# Autodesk Inventor assembly: Topic 15-3_凸輪動力學模擬_test_5
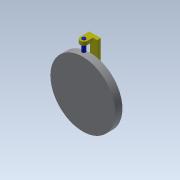
[picture p0: Inventor's stored thumbnail of the model, 180x180]
Saved by Autodesk Inventor 2022 (Build 260153000, 153)
## iProperties
Created: 2020-03-26
Part Number: Topic 15-3_凸輪動力學模擬_test_5
Document SubType Name: Assembly
Designer: Kuan-Lun Hsu
Author: Kuan-Lun Hsu
## Documents named in this file (5)
- C:\Users\Johnny Jou\Documents\GitHub\Special-project\CamSimulaiton\Topic 15-3_凸輪動力學模擬_test_5.iam
- C:\Users\Johnny Jou\Documents\GitHub\Special-project\CamSimulaiton\本體.ipt
- C:\Users\Johnny Jou\Documents\GitHub\Special-project\CamSimulaiton\從動桿.ipt
- C:\Users\Johnny Jou\Documents\GitHub\Special-project\CamSimulaiton\滾輪.ipt
- C:\Users\Johnny Jou\Documents\GitHub\Special-project\CamSimulaiton\凸輪_5.ipt
## Components (4 placed, 4 different names)
1. 本體:1 — 貼合:1, 角度:1, 角度:2, 貼合:2, 角度:3, 貼合:7, 貼合:8
2. 從動桿:1 — 貼合:2, 貼合:3, 角度:3, 貼合:6
3. 滾輪:1 — 貼合:3, 貼合:6
4. 凸輪_5:1 — 貼合:7, 貼合:8
## Relationships (9: Mate 6, Angle 3)
- 貼合:1 [Mate]: 本體:1
- 角度:1 [Angle] (180 deg): 本體:1
- 角度:2 [Angle] (0 deg): 本體:1
- 貼合:2 [Mate]: 本體:1 ↔ 從動桿:1
- 貼合:3 [Mate]: 從動桿:1 ↔ 滾輪:1
- 角度:3 [Angle] (0 deg): 本體:1 ↔ 從動桿:1
- 貼合:6 [Mate]: 從動桿:1 ↔ 滾輪:1
- 貼合:7 [Mate]: 本體:1 ↔ 凸輪_5:1
- 貼合:8 [Mate]: 本體:1 ↔ 凸輪_5:1
